# Autodesk Inventor assembly: poleAssembly
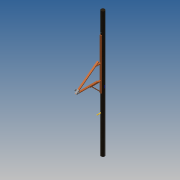
[picture p0: Inventor's stored thumbnail of the model, 180x180]
Saved by Autodesk Inventor 2014 SP1 (Build 180222100, 222)
## iProperties
Created: 2013-12-02
Part Number: poleAssembly
Document SubType Name: Assembly
Designer: Dave
Author: Dave
## Documents named in this file (5)
- C:\Users\Dave\Desktop\hera-cad\support\poleAssembly - OLD.iam
- C:\Users\Dave\Desktop\hera-cad\support\pole.ipt
- C:\Users\Dave\Desktop\hera-cad\support\poleStand.iam
- C:\Users\Dave\Desktop\hera-cad\smallParts\eyebolt_ss_375.ipt
- C:\Users\Dave\Desktop\hera-cad\support\heightMarker.ipt
## Components (4 placed, 4 different names)
1. pole:1 — Mate:1
2. 1m_heightMarker:1 — Mate:1, Mate:2
3. poleStand:1 [sub-assembly] — Mate:2
4. eyebolt_ss_375:1
## Relationships (2: Mate 2)
- Mate:1 (-2143.61 mm): pole:1 ↔ 1m_heightMarker:1
- Mate:2 (1536.7 mm): 1m_heightMarker:1 ↔ poleStand:1
